# Autodesk Inventor assembly: canard_assemb
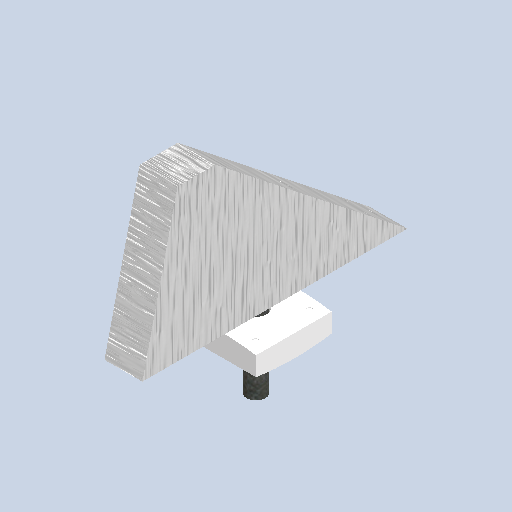
[picture p0: Inventor's stored thumbnail of the model, 512x512]
Saved by Autodesk Inventor 2023 (Build 270158000, 158)
## iProperties
Created: 2023-10-12
Part Number: canard_assemb
Document SubType Name: Assembly
Designer: 310611102
Author: 310611102
## Documents named in this file (6)
- C:\Users\310611102\Documents\Inventor\SSR\avionics_2023ver\assembly\canard_assemb.iam
- C:\Users\310611102\Documents\Inventor\SSR\avionics_2023ver\actuator_system\canard.ipt
- C:\Users\310611102\Documents\Inventor\SSR\avionics_2023ver\actuator_system\gearbox_temp\gearbox_shaft3.ipt
- C:\Users\310611102\Documents\Inventor\SSR\avionics_2023ver\assembly\shift_fixed_socket.ipt
- C:\Users\310611102\Documents\Inventor\SSR\avionics_2023ver\assembly\6000DDU\6000DDU.iam
- C:\Users\310611102\Documents\Inventor\SSR\avionics_2023ver\assembly\FBB4-6_SCM435.ipt
## Components (6 placed, 5 different names)
1. canard:1 — Angle:2
2. gearbox_shaft3:1
3. shift_fixed_socket:1 — Angle:1, Angle:2
4. 6000DDU:1 [sub-assembly]
5. shift_fixed_socket:2 — Angle:1
6. FBB4-6_SCM435:1
## Relationships (8: Insert 3, CylindricalJoint 3, Angle 2)
- [Insert]: shift_fixed_socket:1 ↔ 6000DDU:1
- [Insert]: 6000DDU:1 ↔ shift_fixed_socket:2
- [CylindricalJoint]: gearbox_shaft3:1 ↔ shift_fixed_socket:1
- [CylindricalJoint]: canard:1 ↔ gearbox_shaft3:1
- [Insert]: canard:1 ↔ FBB4-6_SCM435:1
- [CylindricalJoint]: canard:1 ↔ gearbox_shaft3:1
- Angle:1 (0 deg): shift_fixed_socket:1 ↔ shift_fixed_socket:2
- Angle:2 (0 deg): canard:1 ↔ shift_fixed_socket:1
